# Autodesk Inventor assembly: 3-5
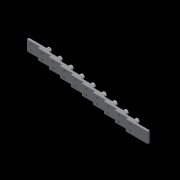
[picture p0: Inventor's stored thumbnail of the model, 180x180]
Saved by Autodesk Inventor 2017 (Build 210142000, 142)
## iProperties
Part Number: 3-5
Material: 一般
Document SubType Name: Assembly
Designer: r0909
Author: r0909
## Documents named in this file (5)
- C:\Users\r0909\Desktop\inventor\3-5.iam
- C:\Users\r0909\Desktop\inventor\3-3.ipt
- C:\Users\r0909\Desktop\inventor\3-4.ipt
- C:\Users\r0909\Desktop\inventor\3-5.1.ipt
- C:\Users\r0909\Desktop\inventor\3-5.2.ipt
## Components (46 placed, 4 different names)
1. 3-3:1 — 貼合:1, 貼合:2, 貼合:3, 貼合:4, 貼合:5, 貼合:6, 貼合:30, 貼合:31, 貼合:52
2. 3-4:1 — 貼合:1, 貼合:2, 貼合:3
3. 3-3:2 — 貼合:4, 貼合:5, 貼合:6, 貼合:7, 貼合:8, 貼合:9, 貼合:53, 貼合:54, 貼合:83
4. 3-3:3 — 貼合:7, 貼合:8, 貼合:9, 貼合:10, 貼合:11, 貼合:12, 貼合:55, 貼合:56, 貼合:84
5. 3-3:4 — 貼合:10, 貼合:11, 貼合:12, 貼合:13, 貼合:14, 貼合:15, 貼合:57, 貼合:58, 貼合:85
6. 3-3:5 — 貼合:13, 貼合:14, 貼合:15, 貼合:16, 貼合:17, 貼合:18, 貼合:59, 貼合:60, 貼合:86
7. 3-3:6 — 貼合:16, 貼合:17, 貼合:18, 貼合:19, 貼合:20, 貼合:21, 貼合:61, 貼合:76, 貼合:87
8. 3-3:7 — 貼合:19, 貼合:20, 貼合:21, 貼合:22, 貼合:23, 貼合:24, 貼合:77, 貼合:78, 貼合:88
9. 3-3:8 — 貼合:22, 貼合:23, 貼合:24, 貼合:25, 貼合:26, 貼合:27, 貼合:79, 貼合:80, 貼合:89
10. 3-3:9 — 貼合:25, 貼合:26, 貼合:27, 貼合:81, 貼合:82, 貼合:90
11. 3-5.1:1 — 貼合:28, 貼合:29, 貼合:30, 角度:1, 齊平:1
12. 3-5.2:1 — 貼合:28, 貼合:29, 貼合:31
13. 3-5.1:2 — 貼合:52, 齊平:1
14. 3-5.2:2
15. 3-5.1:3 — 貼合:53, 齊平:9
16. 3-5.2:3 — 貼合:83
17. 3-5.1:4 — 貼合:54, 齊平:9
18. 3-5.2:4
19. 3-5.1:5 — 貼合:55, 齊平:8
20. 3-5.2:5 — 貼合:84
21. 3-5.1:6 — 貼合:56, 齊平:8
22. 3-5.2:6
23. 3-5.1:7 — 貼合:60, 齊平:6
24. 3-5.2:7
25. 3-5.1:8 — 貼合:61, 齊平:5
26. 3-5.2:8 — 貼合:87
27. 3-5.1:9 — 貼合:59, 齊平:6
28. 3-5.2:9 — 貼合:86
29. 3-5.1:10 — 貼合:58, 齊平:7
30. 3-5.2:10
31. 3-5.1:11 — 貼合:57, 齊平:7
32. 3-5.2:11 — 貼合:85
33. 3-5.1:12 — 貼合:76, 齊平:5
34. 3-5.2:12
35. 3-5.1:13 — 貼合:77, 齊平:4
36. 3-5.2:13 — 貼合:88
37. 3-5.1:14 — 貼合:78, 齊平:4
38. 3-5.2:14
39. 3-5.1:15 — 貼合:79, 齊平:3
40. 3-5.2:15 — 貼合:89
41. 3-5.1:16 — 貼合:80, 齊平:3
42. 3-5.2:16
43. 3-5.1:17 — 貼合:81, 齊平:2
44. 3-5.2:17
45. 3-5.1:18 — 貼合:82, 齊平:2
46. 3-5.2:18 — 貼合:90
## Relationships (100: Mate 90, Flush 9, Angle 1)
- 貼合:1 [Mate]: 3-3:1 ↔ 3-4:1
- 貼合:2 [Mate]: 3-3:1 ↔ 3-4:1
- 貼合:3 [Mate]: 3-3:1 ↔ 3-4:1
- 貼合:4 [Mate]: 3-3:1 ↔ 3-3:2
- 貼合:5 [Mate]: 3-3:1 ↔ 3-3:2
- 貼合:6 [Mate]: 3-3:1 ↔ 3-3:2
- 貼合:7 [Mate]: 3-3:2 ↔ 3-3:3
- 貼合:8 [Mate]: 3-3:2 ↔ 3-3:3
- 貼合:9 [Mate]: 3-3:2 ↔ 3-3:3
- 貼合:10 [Mate]: 3-3:3 ↔ 3-3:4
- 貼合:11 [Mate]: 3-3:3 ↔ 3-3:4
- 貼合:12 [Mate]: 3-3:3 ↔ 3-3:4
- 貼合:13 [Mate]: 3-3:4 ↔ 3-3:5
- 貼合:14 [Mate]: 3-3:4 ↔ 3-3:5
- 貼合:15 [Mate]: 3-3:4 ↔ 3-3:5
- 貼合:16 [Mate]: 3-3:5 ↔ 3-3:6
- 貼合:17 [Mate]: 3-3:5 ↔ 3-3:6
- 貼合:18 [Mate]: 3-3:5 ↔ 3-3:6
- 貼合:19 [Mate]: 3-3:6 ↔ 3-3:7
- 貼合:20 [Mate]: 3-3:6 ↔ 3-3:7
- 貼合:21 [Mate]: 3-3:6 ↔ 3-3:7
- 貼合:22 [Mate]: 3-3:7 ↔ 3-3:8
- 貼合:23 [Mate]: 3-3:7 ↔ 3-3:8
- 貼合:24 [Mate]: 3-3:7 ↔ 3-3:8
- 貼合:25 [Mate]: 3-3:8 ↔ 3-3:9
- 貼合:26 [Mate]: 3-3:8 ↔ 3-3:9
- 貼合:27 [Mate]: 3-3:8 ↔ 3-3:9
- 貼合:28 [Mate]: 3-5.1:1 ↔ 3-5.2:1
- 貼合:29 [Mate]: 3-5.1:1 ↔ 3-5.2:1
- 貼合:30 [Mate]: 3-3:1 ↔ 3-5.1:1
- 貼合:31 [Mate]: 3-3:1 ↔ 3-5.2:1
- 角度:1 [Angle] (0 deg): 3-5.1:1
- [Mate]: 3-5.1:2 ↔ 3-5.2:2
- [Mate]: 3-5.1:2 ↔ 3-5.2:2
- [Mate]: 3-5.1:3 ↔ 3-5.2:3
- [Mate]: 3-5.1:3 ↔ 3-5.2:3
- [Mate]: 3-5.1:4 ↔ 3-5.2:4
- [Mate]: 3-5.1:4 ↔ 3-5.2:4
- [Mate]: 3-5.1:5 ↔ 3-5.2:5
- [Mate]: 3-5.1:5 ↔ 3-5.2:5
- [Mate]: 3-5.1:6 ↔ 3-5.2:6
- [Mate]: 3-5.1:6 ↔ 3-5.2:6
- [Mate]: 3-5.1:7 ↔ 3-5.2:7
- [Mate]: 3-5.1:7 ↔ 3-5.2:7
- [Mate]: 3-5.1:8 ↔ 3-5.2:8
- [Mate]: 3-5.1:8 ↔ 3-5.2:8
- [Mate]: 3-5.1:9 ↔ 3-5.2:9
- [Mate]: 3-5.1:9 ↔ 3-5.2:9
- [Mate]: 3-5.1:10 ↔ 3-5.2:10
- [Mate]: 3-5.1:10 ↔ 3-5.2:10
- [Mate]: 3-5.1:11 ↔ 3-5.2:11
- [Mate]: 3-5.1:11 ↔ 3-5.2:11
- 貼合:52 [Mate]: 3-3:1 ↔ 3-5.1:2
- 齊平:1 [Flush]: 3-5.1:1 ↔ 3-5.1:2
- 貼合:53 [Mate]: 3-3:2 ↔ 3-5.1:3
- 貼合:54 [Mate]: 3-3:2 ↔ 3-5.1:4
- 貼合:55 [Mate]: 3-3:3 ↔ 3-5.1:5
- 貼合:56 [Mate]: 3-3:3 ↔ 3-5.1:6
- 貼合:57 [Mate]: 3-3:4 ↔ 3-5.1:11
- 貼合:58 [Mate]: 3-3:4 ↔ 3-5.1:10
- 貼合:59 [Mate]: 3-3:5 ↔ 3-5.1:9
- 貼合:60 [Mate]: 3-3:5 ↔ 3-5.1:7
- 貼合:61 [Mate]: 3-3:6 ↔ 3-5.1:8
- [Mate]: 3-5.1:12 ↔ 3-5.2:12
- [Mate]: 3-5.1:12 ↔ 3-5.2:12
- [Mate]: 3-5.1:13 ↔ 3-5.2:13
- [Mate]: 3-5.1:13 ↔ 3-5.2:13
- [Mate]: 3-5.1:14 ↔ 3-5.2:14
- [Mate]: 3-5.1:14 ↔ 3-5.2:14
- [Mate]: 3-5.1:15 ↔ 3-5.2:15
- [Mate]: 3-5.1:15 ↔ 3-5.2:15
- [Mate]: 3-5.1:16 ↔ 3-5.2:16
- [Mate]: 3-5.1:16 ↔ 3-5.2:16
- [Mate]: 3-5.1:17 ↔ 3-5.2:17
- [Mate]: 3-5.1:17 ↔ 3-5.2:17
- [Mate]: 3-5.1:18 ↔ 3-5.2:18
- [Mate]: 3-5.1:18 ↔ 3-5.2:18
- 貼合:76 [Mate]: 3-3:6 ↔ 3-5.1:12
- 貼合:77 [Mate]: 3-3:7 ↔ 3-5.1:13
- 貼合:78 [Mate]: 3-3:7 ↔ 3-5.1:14
- 貼合:79 [Mate]: 3-3:8 ↔ 3-5.1:15
- 貼合:80 [Mate]: 3-3:8 ↔ 3-5.1:16
- 貼合:81 [Mate]: 3-3:9 ↔ 3-5.1:17
- 貼合:82 [Mate]: 3-3:9 ↔ 3-5.1:18
- 貼合:83 [Mate]: 3-3:2 ↔ 3-5.2:3
- 貼合:84 [Mate]: 3-3:3 ↔ 3-5.2:5
- 貼合:85 [Mate]: 3-3:4 ↔ 3-5.2:11
- 貼合:86 [Mate]: 3-3:5 ↔ 3-5.2:9
- 貼合:87 [Mate]: 3-3:6 ↔ 3-5.2:8
- 貼合:88 [Mate]: 3-3:7 ↔ 3-5.2:13
- 貼合:89 [Mate]: 3-3:8 ↔ 3-5.2:15
- 貼合:90 [Mate]: 3-3:9 ↔ 3-5.2:18
- 齊平:2 [Flush]: 3-5.1:17 ↔ 3-5.1:18
- 齊平:3 [Flush]: 3-5.1:15 ↔ 3-5.1:16
- 齊平:4 [Flush]: 3-5.1:13 ↔ 3-5.1:14
- 齊平:5 [Flush]: 3-5.1:8 ↔ 3-5.1:12
- 齊平:6 [Flush]: 3-5.1:7 ↔ 3-5.1:9
- 齊平:7 [Flush]: 3-5.1:10 ↔ 3-5.1:11
- 齊平:8 [Flush]: 3-5.1:5 ↔ 3-5.1:6
- 齊平:9 [Flush]: 3-5.1:3 ↔ 3-5.1:4
## Named parameters: d32_d27 = 0 mm, d33_d28 = 0 mm, d34_d27 = 0 mm, d35_d28 = 0 mm, d36_d27 = 0 mm, d37_d28 = 0 mm, d38_d27 = 0 mm, d39_d28 = 0 mm, d40_d27 = 0 mm, d41_d28 = 0 mm, d42_d27 = 0 mm, d43_d28 = 0 mm, d44_d27 = 0 mm, d45_d28 = 0 mm, d46_d27 = 0 mm, d47_d28 = 0 mm, d48_d27 = 0 mm, d49_d28 = 0 mm, d50_d27 = 0 mm, d51_d28 = 0 mm, d63_d27 = 0 mm, d64_d28 = 0 mm, d65_d27 = 0 mm, d66_d28 = 0 mm, d67_d27 = 0 mm, d68_d28 = 0 mm, d69_d27 = 0 mm, d70_d28 = 0 mm, d71_d27 = 0 mm, d72_d28 = 0 mm, d73_d27 = 0 mm, d74_d28 = 0 mm, d75_d27 = 0 mm, d76_d28 = 0 mm
